# Autodesk Inventor assembly: parallel manipulator dummy
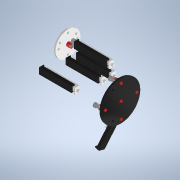
[picture p0: Inventor's stored thumbnail of the model, 180x180]
Saved by Autodesk Inventor 2021 (Build 250183000, 183)
## iProperties
Created: 2022-03-22
Part Number: parallel manipulator dummy
Document SubType Name: Assembly
Designer: techv
Author: techv
## Documents named in this file (8)
- D:\Projects\Major Project\Design\parallel manipulator dummy.iam
- D:\Projects\Major Project\Design\prismatic link inner.ipt
- D:\Projects\Major Project\Design\prismatic link outer.ipt
- D:\Projects\Mini project\parallel manipulator design and fab\3d printing V2\Craftsman Socket U-Joint Base.ipt
- D:\Projects\Mini project\parallel manipulator design and fab\3d printing V2\Craftsman Socket U-Joint Intermediate Body.ipt
- D:\Projects\Mini project\parallel manipulator design and fab\3d printing V2\Craftsman Socket U-Joint Drive.ipt
- D:\Projects\Major Project\Design\Base.ipt
- D:\Projects\Major Project\Design\end effector Plate.ipt
## Components (30 placed, 7 different names)
1. prismatic link inner:1 — Mate:1, Mate:2
2. prismatic link outer:1 — Mate:1, Mate:2
3. Craftsman Socket U-Joint Base:1 — Mate:16, Mate:17, Mate:18
4. Craftsman Socket U-Joint Intermediate Body:1
5. Craftsman Socket U-Joint Drive:1 — Mate:14, Mate:15
6. prismatic link inner:2
7. prismatic link outer:2
8. prismatic link inner:3
9. prismatic link outer:3
10. prismatic link inner:4
11. prismatic link outer:4 — Mate:16, Mate:17, Mate:18
12. prismatic link inner:5
13. prismatic link outer:5
14. Base:1 — Mate:14, Mate:15, Mate:34, Mate:35, Mate:37, Mate:38, Mate:39, Mate:40, Mate:41, Mate:42
15. end effector Plate:1 — Mate:46, Mate:47
16. Craftsman Socket U-Joint Base:2
17. Craftsman Socket U-Joint Intermediate Body:2
18. Craftsman Socket U-Joint Drive:2 — Mate:41, Mate:42
19. Craftsman Socket U-Joint Base:3
20. Craftsman Socket U-Joint Intermediate Body:3
21. Craftsman Socket U-Joint Drive:3 — Mate:39, Mate:40
22. Craftsman Socket U-Joint Base:5
23. Craftsman Socket U-Joint Intermediate Body:5
24. Craftsman Socket U-Joint Drive:5 — Mate:37, Mate:38
25. Craftsman Socket U-Joint Base:6
26. Craftsman Socket U-Joint Intermediate Body:6
27. Craftsman Socket U-Joint Drive:6 — Mate:34, Mate:35
28. Craftsman Socket U-Joint Base:7
29. Craftsman Socket U-Joint Intermediate Body:7
30. Craftsman Socket U-Joint Drive:7 — Mate:46, Mate:47
## Relationships (61: Mate 43, Angle 12, Flush 6)
- Mate:1: prismatic link inner:1 ↔ prismatic link outer:1
- Mate:2: prismatic link inner:1 ↔ prismatic link outer:1
- [Mate]: Craftsman Socket U-Joint Intermediate Body:1 ↔ Craftsman Socket U-Joint Drive:1
- [Mate]: Craftsman Socket U-Joint Base:1 ↔ Craftsman Socket U-Joint Intermediate Body:1
- [Flush]: Craftsman Socket U-Joint Base:1 ↔ Craftsman Socket U-Joint Intermediate Body:1
- [Mate]: Craftsman Socket U-Joint Intermediate Body:1 ↔ Craftsman Socket U-Joint Drive:1
- [Angle] (10 deg): Craftsman Socket U-Joint Base:1 ↔ Craftsman Socket U-Joint Intermediate Body:1
- [Angle] (15 deg): Craftsman Socket U-Joint Intermediate Body:1 ↔ Craftsman Socket U-Joint Drive:1
- [Mate]: prismatic link inner:2 ↔ prismatic link outer:2
- [Mate]: prismatic link inner:2 ↔ prismatic link outer:2
- [Mate]: prismatic link inner:3 ↔ prismatic link outer:3
- [Mate]: prismatic link inner:3 ↔ prismatic link outer:3
- [Mate]: prismatic link inner:4 ↔ prismatic link outer:4
- [Mate]: prismatic link inner:4 ↔ prismatic link outer:4
- [Mate]: prismatic link inner:5 ↔ prismatic link outer:5
- [Mate]: prismatic link inner:5 ↔ prismatic link outer:5
- Mate:14: Craftsman Socket U-Joint Drive:1 ↔ Base:1
- Mate:15: Craftsman Socket U-Joint Drive:1 ↔ Base:1
- Mate:16: Craftsman Socket U-Joint Base:1 ↔ prismatic link outer:4
- Mate:17: Craftsman Socket U-Joint Base:1 ↔ prismatic link outer:4
- Mate:18: Craftsman Socket U-Joint Base:1 ↔ prismatic link outer:4
- [Mate]: Craftsman Socket U-Joint Intermediate Body:2 ↔ Craftsman Socket U-Joint Drive:2
- [Mate]: Craftsman Socket U-Joint Base:2 ↔ Craftsman Socket U-Joint Intermediate Body:2
- [Flush]: Craftsman Socket U-Joint Base:2 ↔ Craftsman Socket U-Joint Intermediate Body:2
- [Mate]: Craftsman Socket U-Joint Intermediate Body:2 ↔ Craftsman Socket U-Joint Drive:2
- [Angle] (10 deg): Craftsman Socket U-Joint Base:2 ↔ Craftsman Socket U-Joint Intermediate Body:2
- [Angle] (15 deg): Craftsman Socket U-Joint Intermediate Body:2 ↔ Craftsman Socket U-Joint Drive:2
- [Mate]: Craftsman Socket U-Joint Intermediate Body:3 ↔ Craftsman Socket U-Joint Drive:3
- [Mate]: Craftsman Socket U-Joint Base:3 ↔ Craftsman Socket U-Joint Intermediate Body:3
- [Flush]: Craftsman Socket U-Joint Base:3 ↔ Craftsman Socket U-Joint Intermediate Body:3
- [Mate]: Craftsman Socket U-Joint Intermediate Body:3 ↔ Craftsman Socket U-Joint Drive:3
- [Angle] (10 deg): Craftsman Socket U-Joint Base:3 ↔ Craftsman Socket U-Joint Intermediate Body:3
- [Angle] (15 deg): Craftsman Socket U-Joint Intermediate Body:3 ↔ Craftsman Socket U-Joint Drive:3
- [Mate]: Craftsman Socket U-Joint Intermediate Body:5 ↔ Craftsman Socket U-Joint Drive:5
- [Mate]: Craftsman Socket U-Joint Base:5 ↔ Craftsman Socket U-Joint Intermediate Body:5
- [Flush]: Craftsman Socket U-Joint Base:5 ↔ Craftsman Socket U-Joint Intermediate Body:5
- [Mate]: Craftsman Socket U-Joint Intermediate Body:5 ↔ Craftsman Socket U-Joint Drive:5
- [Angle] (10 deg): Craftsman Socket U-Joint Base:5 ↔ Craftsman Socket U-Joint Intermediate Body:5
- [Angle] (15 deg): Craftsman Socket U-Joint Intermediate Body:5 ↔ Craftsman Socket U-Joint Drive:5
- [Mate]: Craftsman Socket U-Joint Intermediate Body:6 ↔ Craftsman Socket U-Joint Drive:6
- [Mate]: Craftsman Socket U-Joint Base:6 ↔ Craftsman Socket U-Joint Intermediate Body:6
- [Flush]: Craftsman Socket U-Joint Base:6 ↔ Craftsman Socket U-Joint Intermediate Body:6
- [Mate]: Craftsman Socket U-Joint Intermediate Body:6 ↔ Craftsman Socket U-Joint Drive:6
- [Angle] (10 deg): Craftsman Socket U-Joint Base:6 ↔ Craftsman Socket U-Joint Intermediate Body:6
- [Angle] (15 deg): Craftsman Socket U-Joint Intermediate Body:6 ↔ Craftsman Socket U-Joint Drive:6
- Mate:34: Base:1 ↔ Craftsman Socket U-Joint Drive:6
- Mate:35: Base:1 ↔ Craftsman Socket U-Joint Drive:6
- Mate:37: Base:1 ↔ Craftsman Socket U-Joint Drive:5
- Mate:38: Base:1 ↔ Craftsman Socket U-Joint Drive:5
- Mate:39: Base:1 ↔ Craftsman Socket U-Joint Drive:3
- Mate:40: Base:1 ↔ Craftsman Socket U-Joint Drive:3
- Mate:41: Base:1 ↔ Craftsman Socket U-Joint Drive:2
- Mate:42: Base:1 ↔ Craftsman Socket U-Joint Drive:2
- [Mate]: Craftsman Socket U-Joint Intermediate Body:7 ↔ Craftsman Socket U-Joint Drive:7
- [Mate]: Craftsman Socket U-Joint Base:7 ↔ Craftsman Socket U-Joint Intermediate Body:7
- [Flush]: Craftsman Socket U-Joint Base:7 ↔ Craftsman Socket U-Joint Intermediate Body:7
- [Mate]: Craftsman Socket U-Joint Intermediate Body:7 ↔ Craftsman Socket U-Joint Drive:7
- [Angle] (10 deg): Craftsman Socket U-Joint Base:7 ↔ Craftsman Socket U-Joint Intermediate Body:7
- [Angle] (15 deg): Craftsman Socket U-Joint Intermediate Body:7 ↔ Craftsman Socket U-Joint Drive:7
- Mate:46: end effector Plate:1 ↔ Craftsman Socket U-Joint Drive:7
- Mate:47: end effector Plate:1 ↔ Craftsman Socket U-Joint Drive:7
## Named parameters: d282_d185_d165_d90_d0 = 0 mm, d283_d186_d166_d1 = 0 mm, d284_d187_d167_d92_d11 = 165 deg, d285_d188_d168_d93_d12 = 15 deg, d286_d189_d169_d13 = 15 deg, d287_d190_d170_d14 = 165 deg, d288_d191_d171_d15 = 15 deg, d289_d192_d172_d97_d2 = 0 mm, d290_d193_d173_d98_d3 = 0 mm, d291_d194_d174_d99_d4 = 10 deg, d19_d0 = 0 mm, d20_d1 = 0 mm, d21_d0 = 0 mm, d22_d1 = 0 mm, d23_d0 = 0 mm, d24_d1 = 0 mm, d25_d0 = 0 mm, d26_d1 = 0 mm, d32_d282_d185_d165_d90_d0 = 0 mm, d33_d283_d186_d166_d1 = 0 mm, d34_d284_d187_d167_d92_d11 = 165 deg, d35_d285_d188_d168_d93_d12 = 15 deg, d36_d286_d189_d169_d13 = 15 deg, d37_d287_d190_d170_d14 = 165 deg, d38_d288_d191_d171_d15 = 15 deg, d39_d289_d192_d172_d97_d2 = 0 mm, d40_d290_d193_d173_d98_d3 = 0 mm, d41_d291_d194_d174_d99_d4 = 10 deg, d48_d282_d185_d165_d90_d0 = 0 mm, d49_d283_d186_d166_d1 = 0 mm, d50_d284_d187_d167_d92_d11 = 165 deg, d51_d285_d188_d168_d93_d12 = 15 deg, d52_d286_d189_d169_d13 = 15 deg, d53_d287_d190_d170_d14 = 165 deg, d54_d288_d191_d171_d15 = 15 deg, d55_d289_d192_d172_d97_d2 = 0 mm, d56_d290_d193_d173_d98_d3 = 0 mm, d57_d291_d194_d174_d99_d4 = 10 deg, d80_d282_d185_d165_d90_d0 = 0 mm, d81_d283_d186_d166_d1 = 0 mm, d82_d284_d187_d167_d92_d11 = 165 deg, d83_d285_d188_d168_d93_d12 = 15 deg, d84_d286_d189_d169_d13 = 15 deg, d85_d287_d190_d170_d14 = 165 deg, d86_d288_d191_d171_d15 = 15 deg, d87_d289_d192_d172_d97_d2 = 0 mm, d88_d290_d193_d173_d98_d3 = 0 mm, d89_d291_d194_d174_d99_d4 = 10 deg, d96_d282_d185_d165_d90_d0 = 0 mm, d97_d283_d186_d166_d1 = 0 mm, d98_d284_d187_d167_d92_d11 = 165 deg, d99_d285_d188_d168_d93_d12 = 15 deg, d100_d286_d189_d169_d13 = 15 deg, d101_d287_d190_d170_d14 = 165 deg, d102_d288_d191_d171_d15 = 15 deg, d103_d289_d192_d172_d97_d2 = 0 mm, d104_d290_d193_d173_d98_d3 = 0 mm, d105_d291_d194_d174_d99_d4 = 10 deg, d121_d48_d282_d185_d165_d90_d0 = 0 mm, d122_d49_d283_d186_d166_d1 = 0 mm, d123_d50_d284_d187_d167_d92_d11 = 165 deg, d124_d51_d285_d188_d168_d93_d12 = 15 deg, d125_d52_d286_d189_d169_d13 = 15 deg, d126_d53_d287_d190_d170_d14 = 165 deg, d127_d54_d288_d191_d171_d15 = 15 deg, d128_d55_d289_d192_d172_d97_d2 = 0 mm, d129_d56_d290_d193_d173_d98_d3 = 0 mm, d130_d57_d291_d194_d174_d99_d4 = 10 deg
